# Autodesk Inventor assembly: Actuator
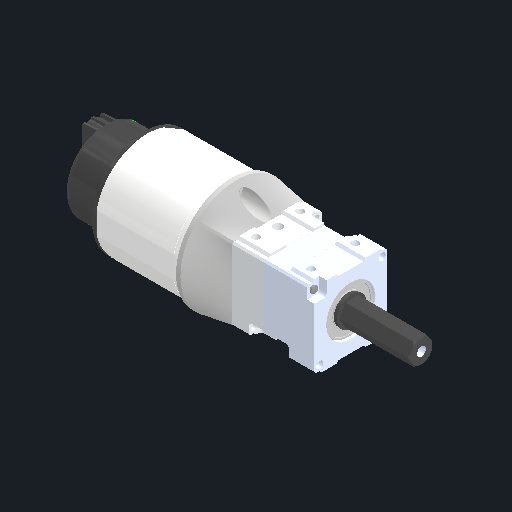
[picture p0: Inventor's stored thumbnail of the model, 512x512]
Saved by Autodesk Inventor 2023 (Build 270158000, 158)
## iProperties
Created: 2022-05-02
Part Number: Actuator
Document SubType Name: Assembly
Designer: FizzyApple12
Author: FizzyApple12
## Documents named in this file (5)
- C:\Users\FizzyApple12\Desktop\Ping Pong Robot\Actuator.iam
- C:\Users\FizzyApple12\Desktop\Ping Pong Robot\OTS\vex-pro\versaplanetary\VersaPlanetary v2 Single Stage 10 1 with BAG .ipt
- C:\Users\FizzyApple12\Desktop\Ping Pong Robot\OTS\vex-pro\versaplanetary\VersaPlanetary CIM Adapter (217-4018).ipt
- C:\Users\FizzyApple12\Desktop\Ping Pong Robot\OTS\vex-pro\versaplanetary\VP Press On Motor Coupler (Falcon Motor) (217-6789).ipt
- C:\Users\FizzyApple12\Desktop\Ping Pong Robot\OTS\vex-pro\Falcon 500, Powered by Talon FX (217-6515) No Shaft.ipt
## Components (4 placed, 4 different names)
1. VersaPlanetary v2 Single Stage 10 1 with BAG :1 — Mate:1, Mate:2, Mate:3, Mate:4
2. VersaPlanetary CIM Adapter (217-4018):1 — Mate:1, Mate:2, Mate:5, Mate:6, Mate:7
3. VP Press On Motor Coupler (Falcon Motor) (217-6789):1 — Mate:3, Mate:4
4. Falcon 500, Powered by Talon FX (217-6515) No Shaft:1 — Mate:5, Mate:6, Mate:7
## Relationships (7: Mate 7)
- Mate:1: VersaPlanetary v2 Single Stage 10 1 with BAG :1 ↔ VersaPlanetary CIM Adapter (217-4018):1
- Mate:2: VersaPlanetary v2 Single Stage 10 1 with BAG :1 ↔ VersaPlanetary CIM Adapter (217-4018):1
- Mate:3: VersaPlanetary v2 Single Stage 10 1 with BAG :1 ↔ VP Press On Motor Coupler (Falcon Motor) (217-6789):1
- Mate:4: VersaPlanetary v2 Single Stage 10 1 with BAG :1 ↔ VP Press On Motor Coupler (Falcon Motor) (217-6789):1
- Mate:5: VersaPlanetary CIM Adapter (217-4018):1 ↔ Falcon 500, Powered by Talon FX (217-6515) No Shaft:1
- Mate:6: VersaPlanetary CIM Adapter (217-4018):1 ↔ Falcon 500, Powered by Talon FX (217-6515) No Shaft:1
- Mate:7: VersaPlanetary CIM Adapter (217-4018):1 ↔ Falcon 500, Powered by Talon FX (217-6515) No Shaft:1
